# Autodesk Inventor assembly: PAS614L-VL3
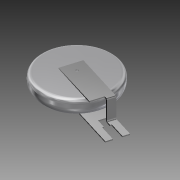
[picture p0: Inventor's stored thumbnail of the model, 180x180]
Saved by Autodesk Inventor 2014 (Build 180170000, 170)
## iProperties
Created: 2014-11-22
Part Number: PAS614L-VL3
Document SubType Name: Assembly
Designer: DV
Author: DV
## Documents named in this file (4)
- C:\Users\DV\Documents\github\Disceep\PAS614L-VL3.iam
- C:\Users\DV\Documents\github\Disceep\SuperCap_PAS614L.ipt
- C:\Users\DV\Documents\github\Disceep\PosTerm.ipt
- C:\Users\DV\Documents\github\Disceep\NegTerm.ipt
## Components (3 placed, 3 different names)
1. SuperCap_PAS614L:1 — Mate:1
2. PosTerm:1 — Flush:1, Flush:2, Mate:1, Mate:2
3. NegTerm:1 — Flush:1, Flush:2
## Relationships (4: Flush 2, Mate 2)
- Flush:1: PosTerm:1 ↔ NegTerm:1
- Flush:2: PosTerm:1 ↔ NegTerm:1
- Mate:1: SuperCap_PAS614L:1 ↔ PosTerm:1
- Mate:2: PosTerm:1
